# Autodesk Inventor assembly: Assembly
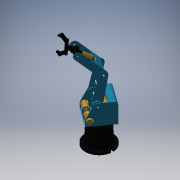
[picture p0: Inventor's stored thumbnail of the model, 180x180]
Saved by Autodesk Inventor 2016 (Build 200138000, 138)
## iProperties
Created: 2015-05-19
Part Number: Assembly
Document SubType Name: Assembly
Designer: CHUNGBK
Author: CHUNGBK
## Documents named in this file (9)
- C:\Users\jonathan\Desktop\Five Axis Serial Robotic Arm\Inventor\Scorbot Complete Assembly.iam
- C:\Users\jonathan\Desktop\Five Axis Serial Robotic Arm\Inventor\Scorbot Platform.iam
- C:\Users\jonathan\Desktop\Five Axis Serial Robotic Arm\Inventor\Scorbot Shoulder.iam
- C:\Users\jonathan\Desktop\Five Axis Serial Robotic Arm\Inventor\Scorbot Elbow.iam
- C:\Users\jonathan\Desktop\Five Axis Serial Robotic Arm\Inventor\Motor Shaft.ipt
- C:\Users\jonathan\Desktop\Five Axis Serial Robotic Arm\Inventor\Bevel Gear.ipt
- C:\Users\jonathan\Desktop\Five Axis Serial Robotic Arm\Inventor\Gripper Gear.ipt
- C:\Users\jonathan\Desktop\Five Axis Serial Robotic Arm\Inventor\Gripper Motor.ipt
- C:\Users\jonathan\Desktop\Five Axis Serial Robotic Arm\Inventor\Base.ipt
## Components (14 placed, 7 different names)
1. Scorbot Platform:1 [sub-assembly] — Mate:1, Mate:2, Mate:4, Mate:5, Mate:6, Mate:7, Mate:8, Mate:9, Mate:10, Mate:11, Mate:12, Mate:13, Flush:6, Mate:24, Angle:3, Angle:4, Angle:5, Angle:6, Angle:7, Mate:25, Mate:26
2. Scorbot Shoulder:1 [sub-assembly] — Mate:1, Mate:2, Mate:3, Flush:5, Angle:4
3. Scorbot Elbow:1 [sub-assembly] — Mate:3, Flush:5, Mate:14, Mate:15, Mate:16, Angle:1, Angle:2, Angle:5
4. Motor Shaft:1 — Mate:4, Mate:5
5. Motor Shaft:2 — Mate:7, Mate:12
6. Motor Shaft:3 — Mate:8, Mate:13
7. Motor Shaft:4 — Mate:9, Mate:10
8. Motor Shaft:5 — Mate:6, Mate:11
9. Bevel Gear1:1 — Mate:16, Mate:19, Rotation:2
10. Bevel Gear1:4 — Mate:18, Mate:19, Rotation:1, Rotation:2, Angle:1, Mate:20, Mate:21, Angle:6, Angle:7
11. Bevel Gear1:3 — Mate:14, Mate:15, Mate:18, Rotation:1
12. Gripper Motor:1 — Mate:22, Mate:23, Angle:2
13. Motor Shaft:6 — Mate:20, Mate:21, Mate:22, Mate:23
14. Base:1 — Mate:25, Mate:26
## Relationships (36: Mate 25, Angle 7, Flush 2, RelateRotation 2)
- Mate:1: Scorbot Platform:1 ↔ Scorbot Shoulder:1
- Mate:2 (23.3997 mm): Scorbot Platform:1 ↔ Scorbot Shoulder:1
- Mate:3: Scorbot Shoulder:1 ↔ Scorbot Elbow:1
- Flush:5 (8.7313 mm): Scorbot Shoulder:1 ↔ Scorbot Elbow:1
- Mate:4: Scorbot Platform:1 ↔ Motor Shaft:1
- Mate:5 (-19.05 mm): Scorbot Platform:1 ↔ Motor Shaft:1
- Mate:6: Scorbot Platform:1 ↔ Motor Shaft:5
- Mate:7: Scorbot Platform:1 ↔ Motor Shaft:2
- Mate:8: Scorbot Platform:1 ↔ Motor Shaft:3
- Mate:9: Scorbot Platform:1 ↔ Motor Shaft:4
- Mate:10 (-19.05 mm): Scorbot Platform:1 ↔ Motor Shaft:4
- Mate:11 (19.05 mm): Scorbot Platform:1 ↔ Motor Shaft:5
- Mate:12 (-19.05 mm): Scorbot Platform:1 ↔ Motor Shaft:2
- Mate:13 (-19.05 mm): Scorbot Platform:1 ↔ Motor Shaft:3
- Mate:14: Scorbot Elbow:1 ↔ Bevel Gear1:3
- Mate:15: Scorbot Elbow:1 ↔ Bevel Gear1:3
- Mate:16: Scorbot Elbow:1 ↔ Bevel Gear1:1
- Mate:18: Bevel Gear1:4 ↔ Bevel Gear1:3
- Mate:19: Bevel Gear1:1 ↔ Bevel Gear1:4
- Rotation:1 [RelateRotation] (1 ul): Bevel Gear1:4 ↔ Bevel Gear1:3
- Rotation:2 [RelateRotation] (1 ul): Bevel Gear1:1 ↔ Bevel Gear1:4
- Angle:1 (90 deg): Scorbot Elbow:1 ↔ Bevel Gear1:4
- Mate:20: Bevel Gear1:4 ↔ Motor Shaft:6
- Mate:21: Bevel Gear1:4 ↔ Motor Shaft:6
- Mate:22: Gripper Motor:1 ↔ Motor Shaft:6
- Mate:23: Gripper Motor:1 ↔ Motor Shaft:6
- Angle:2 (0 deg): Scorbot Elbow:1 ↔ Gripper Motor:1
- Flush:6: Scorbot Platform:1
- Mate:24: Scorbot Platform:1
- Angle:3 (180 deg): Scorbot Platform:1
- Angle:4 (0 deg): Scorbot Platform:1 ↔ Scorbot Shoulder:1
- Angle:5 (0 deg): Scorbot Platform:1 ↔ Scorbot Elbow:1
- Angle:6 (0 deg): Scorbot Platform:1 ↔ Bevel Gear1:4
- Angle:7 (0 deg): Scorbot Platform:1 ↔ Bevel Gear1:4
- Mate:25 (23.8252 mm): Scorbot Platform:1 ↔ Base:1
- Mate:26: Scorbot Platform:1 ↔ Base:1
